# Autodesk Inventor assembly: Quad-Load-Cell-Amplifier-to-RS-485-Conv-Module-UpperCover
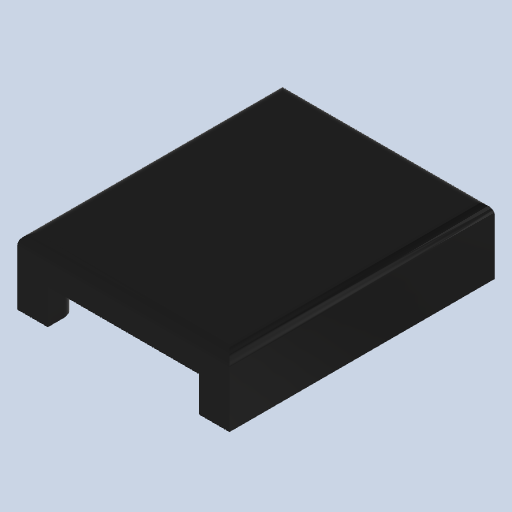
[picture p0: Inventor's stored thumbnail of the model, 512x512]
Saved by Autodesk Inventor 2022.5 (Build 265521000, 521)
## iProperties
Created: 2023-05-09
Part Number: Quad-Load-Cell-Amplifier-to-RS-485-Conv-Module-UpperCover
Document SubType Name: Assembly
Designer: Masato Kubotera
Author: Masato Kubotera
## Documents named in this file (3)
- C:\Users\Masato\Documents\Inventor\SUSTAINA-OP\ModelingFiles\LowerBody\Foot\Quad-Load-Cell-Amplifier-to-RS-485-Conv-Module-UpperCover.iam
- C:\Users\Masato\Documents\Inventor\SUSTAINA-OP\ModelingFiles\LowerBody\Foot\Quad-Load-Cell-Amplifier-to-RS-485-Conv-Module-UpperCover.ipt
- C:\Users\Masato\Documents\Inventor\SUSTAINA-OP\ModelingFiles\COTS\InsertNut\UD-43040.ipt
## Components (5 placed, 2 different names)
1. Quad-Load-Cell-Amplifier-to-RS-485-Conv-Module-UpperCover:1 — フラッシュ:1, フラッシュ:2, フラッシュ:3, 挿入:1, 挿入:2, 挿入:3, 挿入:4
2. UD-43040:1 — 挿入:1
3. UD-43040:2 — 挿入:2
4. UD-43040:3 — 挿入:3
5. UD-43040:4 — 挿入:4
## Relationships (7: Insert 4, Flush 3)
- フラッシュ:1 [Flush]: Quad-Load-Cell-Amplifier-to-RS-485-Conv-Module-UpperCover:1
- フラッシュ:2 [Flush]: Quad-Load-Cell-Amplifier-to-RS-485-Conv-Module-UpperCover:1
- フラッシュ:3 [Flush]: Quad-Load-Cell-Amplifier-to-RS-485-Conv-Module-UpperCover:1
- 挿入:1 [Insert]: Quad-Load-Cell-Amplifier-to-RS-485-Conv-Module-UpperCover:1 ↔ UD-43040:1
- 挿入:2 [Insert]: Quad-Load-Cell-Amplifier-to-RS-485-Conv-Module-UpperCover:1 ↔ UD-43040:2
- 挿入:3 [Insert]: Quad-Load-Cell-Amplifier-to-RS-485-Conv-Module-UpperCover:1 ↔ UD-43040:3
- 挿入:4 [Insert]: Quad-Load-Cell-Amplifier-to-RS-485-Conv-Module-UpperCover:1 ↔ UD-43040:4
